# Autodesk Inventor assembly: auger_assy
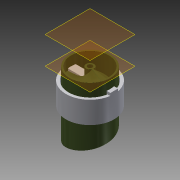
[picture p0: Inventor's stored thumbnail of the model, 180x180]
Saved by Autodesk Inventor 2014 SP2 (Build 180246200, 246)
## iProperties
Created: 2016-03-11
Part Number: auger_assy
Document SubType Name: Assembly
Designer: schrluka
Author: schrluka
## Documents named in this file (3)
- C:\schrluka\private\BarBot\Conception\Mechanical\Ice_Dispenser\auger\auger_assy.iam
- C:\schrluka\private\BarBot\Conception\Mechanical\Ice_Dispenser\auger\auger_element.ipt
- C:\schrluka\private\BarBot\Conception\Mechanical\Ice_Dispenser\auger\tunnel.ipt
## Components (3 placed, 2 different names)
1. auger_element:1 — Mate:1, Mate:2, Flush:1
2. auger_element:2 — Mate:1, Mate:2
3. tunnel:1 — Flush:1
## Relationships (3: Mate 2, Flush 1)
- Mate:1: auger_element:1 ↔ auger_element:2
- Mate:2: auger_element:1 ↔ auger_element:2
- Flush:1: auger_element:1 ↔ tunnel:1
